# Autodesk Inventor assembly: assembly1pt0
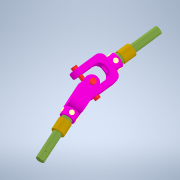
[picture p0: Inventor's stored thumbnail of the model, 180x180]
Saved by Autodesk Inventor 2022 (Build 260153000, 153)
## iProperties
Created: 2023-03-08
Part Number: assembly1pt0
Document SubType Name: Assembly
Designer: karee
Author: karee
## Documents named in this file (12)
- C:\Users\karee\OneDrive\Desktop\UniversalJoint\assembly1pt0.iam
- C:\Users\karee\OneDrive\Desktop\UniversalJoint\shaft.ipt
- C:\Users\karee\OneDrive\Desktop\UniversalJoint\fork.ipt
- C:\Users\karee\OneDrive\Desktop\UniversalJoint\bush.ipt
- C:\Users\karee\OneDrive\Desktop\UniversalJoint\pin.ipt
- C:\Users\karee\OneDrive\Desktop\UniversalJoint\bolt.ipt
- C:\Users\karee\OneDrive\Desktop\UniversalJoint\nut.ipt
- C:\Users\karee\OneDrive\Desktop\UniversalJoint\shaft_MIR.ipt
- C:\Users\karee\OneDrive\Desktop\UniversalJoint\fork_MIR.ipt
- C:\Users\karee\OneDrive\Desktop\UniversalJoint\bush_MIR.ipt
- C:\Users\karee\OneDrive\Desktop\UniversalJoint\pin_MIR.ipt
- C:\Users\karee\OneDrive\Desktop\UniversalJoint\bolt_MIR.ipt
## Components (19 placed, 11 different names)
1. shaft:1 — Rigid:1, Rotational:1, Angle:2
2. fork:1 — Rigid:1, Rigid:2, Rigid:3, Mate:2, Mate:3
3. bush:1 — Rotational:1
4. nut:1 — Rotational:2, Mate:1, Rotational:4, Mate:7
5. shaft_MIR:1 — Rigid:4, Rotational:3, Angle:2
6. fork_MIR:1 — Mate:4, Mate:5, Rigid:4, Rigid:5, Rigid:6, Mate:6
7. bush_MIR:1 — Rotational:3
8. pin:1 — Rigid:2
9. pin:2
10. pin:3
11. pin:4
12. bolt:1 — Rigid:3, Rotational:2
13. bolt:2
14. bolt_MIR:1 — Rigid:6, Rotational:4
15. bolt_MIR:2
16. pin_MIR:1 — Rigid:5
17. pin_MIR:2
18. pin_MIR:3
19. pin_MIR:4
## Component patterns: (4 elements, first: pin:1), (2 elements, first: bolt:1), (2 elements, first: bolt_MIR:1), (4 elements, first: pin_MIR:1)
## Relationships (20: Mate 7, WeldJoint 6, RevoluteJoint 4, Angle 2, Flush 1)
- Rigid:1 [WeldJoint]: shaft:1 ↔ fork:1
- Rotational:1 [RevoluteJoint]: shaft:1 ↔ bush:1
- Rigid:2 [WeldJoint]: fork:1 ↔ pin:1
- Rigid:3 [WeldJoint]: fork:1 ↔ bolt:1
- Rotational:2 [RevoluteJoint] (-8.5 mm): nut:1 ↔ bolt:1
- Mate:1: nut:1
- Mate:2: fork:1
- Mate:3: fork:1
- Angle:1 (0 deg)
- Flush:1 (-58.7375 mm)
- Mate:4: fork_MIR:1
- Mate:5: fork_MIR:1
- Rigid:4 [WeldJoint]: shaft_MIR:1 ↔ fork_MIR:1
- Rotational:3 [RevoluteJoint]: shaft_MIR:1 ↔ bush_MIR:1
- Rigid:5 [WeldJoint]: fork_MIR:1 ↔ pin_MIR:1
- Rigid:6 [WeldJoint]: fork_MIR:1 ↔ bolt_MIR:1
- Rotational:4 [RevoluteJoint] (-8.5 mm): nut:1 ↔ bolt_MIR:1
- Mate:6: fork_MIR:1
- Mate:7: nut:1
- Angle:2 (20 deg): shaft:1 ↔ shaft_MIR:1
